# Autodesk Inventor assembly: TwoLegSegemnt_Adaptive
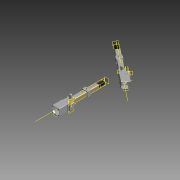
[picture p0: Inventor's stored thumbnail of the model, 180x180]
Saved by Autodesk Inventor 2012 (Build 160160000, 160)
## iProperties
Created: 2011-10-31
Part Number: TwoLegSegemnt_Adaptive
Document SubType Name: Assembly
Designer: KuttaA
Author: KuttaA
## Documents named in this file (2)
- C:\Users\akutta\Dropbox\Hexapod Research\Leg Design\TwoLegSegemnt_Adaptive.iam
- C:\Users\akutta\Dropbox\Hexapod Research\Leg Design\ExtendingArm_ProperConstraints.iam
## Components (2 placed, 1 different names)
1. ExtendingArm_ProperConstraints:1 [sub-assembly] — Mate:1, Flush:2
2. ExtendingArm_ProperConstraints:2 [sub-assembly] — Flush:2
## Relationships (2: Mate 1, Flush 1)
- Mate:1: ExtendingArm_ProperConstraints:1
- Flush:2: ExtendingArm_ProperConstraints:1 ↔ ExtendingArm_ProperConstraints:2
